# Autodesk Inventor assembly: CCM_Mount_AB
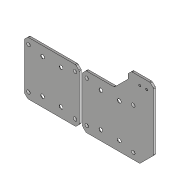
[picture p0: Inventor's stored thumbnail of the model, 180x180]
Saved by Autodesk Inventor 2020 (Build 240168000, 168)
## iProperties
Created: 2021-07-28
Part Number: CCM_Mount_AB
Document SubType Name: Assembly
Designer: magnarecta
Author: magnarecta
## Documents named in this file (3)
- C:\Users\lvglv\Documents\GitHub\Eto_Project\Hardware\Parts\Meviy\Meviy_Asem\CCM_Mount_AB.iam
- C:\Users\lvglv\Documents\GitHub\Eto_Project\Hardware\Parts\Meviy\CCM_Mount_A.ipt
- C:\Users\lvglv\Documents\GitHub\Eto_Project\Hardware\Parts\Meviy\CCM_Mount_B.ipt
## Components (2 placed, 2 different names)
1. CCM_Mount_A:1 — フラッシュ:1, フラッシュ:2, メイト:1
2. CCM_Mount_B:1 — フラッシュ:1, フラッシュ:2, メイト:1
## Relationships (3: Flush 2, Mate 1)
- フラッシュ:1 [Flush]: CCM_Mount_A:1 ↔ CCM_Mount_B:1
- フラッシュ:2 [Flush]: CCM_Mount_A:1 ↔ CCM_Mount_B:1
- メイト:1 [Mate] (5 mm): CCM_Mount_A:1 ↔ CCM_Mount_B:1
